# Autodesk Inventor assembly: boe bot assembly
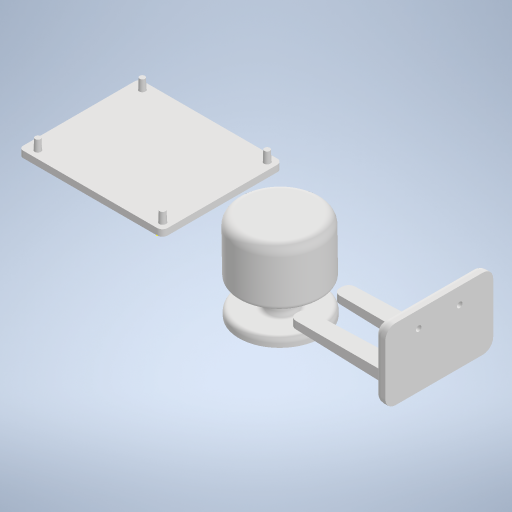
[picture p0: Inventor's stored thumbnail of the model, 512x512]
Saved by Autodesk Inventor 2023.1 (Build 271208000, 208)
## iProperties
Created: 2022-11-17
Part Number: boe bot assembly
Document SubType Name: Assembly
Designer: techv
Author: techv
## Documents named in this file (4)
- D:\Projects\P_boebot\design\boe bot assembly.iam
- D:\Projects\P_boebot\design\pallet holder.ipt
- D:\Projects\P_boebot\design\pallet.ipt
- D:\Projects\P_Telemetry Robot\rapi mount.ipt
## Components (3 placed, 3 different names)
1. pallet holder:1 — Mate:1
2. pallet:1 — Mate:1
3. rapi mount:1
## Relationships (1: Mate 1)
- Mate:1: pallet holder:1 ↔ pallet:1
